# Autodesk Inventor assembly: Low Free Horn
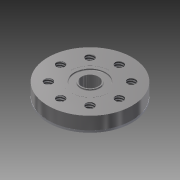
[picture p0: Inventor's stored thumbnail of the model, 180x180]
Saved by Autodesk Inventor 2013 (Build 170138000, 138)
## iProperties
Created: 2014-05-10
Part Number: Low Free Horn
Document SubType Name: Assembly
Designer: andou
Mass: 3.09576 g
Surface Area: 17.9488 cm^2
Volume: 0.966088 cm^3
Density: 3.20443 g/cm^3
Author: andou
## Documents named in this file (5)
- C:\Users\andou\Documents\Inventor\RoboticsProject\project_4\Robot\Free_Horn\Low Free Horn.iam
- C:\Users\andou\Documents\Inventor\RoboticsProject\project_4\Robot\Free_Horn\Bearing Holder.ipt
- C:\Users\andou\Documents\Inventor\RoboticsProject\project_4\Robot\Free_Horn\Bearing.ipt
- C:\Users\andou\Documents\Inventor\RoboticsProject\project_4\Robot\Free_Horn\Acetal_Washer(t0.5).ipt
- C:\Users\andou\Documents\Inventor\RoboticsProject\project_4\Robot\Free_Horn\Bearing_Washer(t0.5).ipt
## Components (4 placed, 4 different names)
1. Bearing Holder:1 — 挿入:1
2. Bearing:1 — 挿入:1, 挿入:2
3. Acetal_Washer(t0.5):1 — 挿入:3
4. Bearing_Washer(t0.5):1 — 挿入:2, 挿入:3
## Relationships (3: Insert 3)
- 挿入:1 [Insert]: Bearing Holder:1 ↔ Bearing:1
- 挿入:2 [Insert]: Bearing:1 ↔ Bearing_Washer(t0.5):1
- 挿入:3 [Insert]: Acetal_Washer(t0.5):1 ↔ Bearing_Washer(t0.5):1
